# Autodesk Inventor assembly: DisceepXL
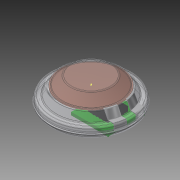
[picture p0: Inventor's stored thumbnail of the model, 180x180]
Saved by Autodesk Inventor 2014 (Build 180170000, 170)
## iProperties
Created: 2014-11-22
Part Number: DisceepXL
Document SubType Name: Assembly
Designer: DV
Author: DV
## Documents named in this file (8)
- C:\Users\DV\Documents\github\Disceep\DisceepXL.iam
- C:\Users\DV\Documents\github\Disceep\PAS614L-VL3.iam
- C:\Users\DV\Documents\github\Disceep\DisceepXL_PCB.ipt
- C:\Users\DV\Documents\github\Disceep\QFN16_4mmx4mm.ipt
- C:\Users\DV\Documents\github\Disceep\DisceepXL_Case.ipt
- C:\Users\DV\Documents\github\Disceep\12mmPiezo.ipt
- C:\Users\DV\Documents\github\Disceep\DisceepSL_CaseBottom.ipt
- C:\Users\DV\Documents\github\Disceep\Part3.ipt
## Components (7 placed, 7 different names)
1. PAS614L-VL3:1 [sub-assembly] — Mate:2, Mate:3, Mate:8
2. DisceepXL_PCB:1 — Mate:1, Mate:2, Mate:3, Mate:7, Mate:9, Angle:1
3. QFN16_4mmx4mm:1 — Mate:1, Flush:7, Mate:7
4. DisceepXL_Case:1 — Flush:9
5. 12mmPiezo:1 — Mate:4, Flush:6, Flush:7
6. DisceepSL_CaseBottom:1 — Flush:8
7. Part3:2 — Flush:9, Angle:1
## Relationships (12: Mate 7, Flush 4, Angle 1)
- Mate:1: DisceepXL_PCB:1 ↔ QFN16_4mmx4mm:1
- Mate:2: PAS614L-VL3:1 ↔ DisceepXL_PCB:1
- Mate:3 (0.254 mm): PAS614L-VL3:1 ↔ DisceepXL_PCB:1
- Mate:4: 12mmPiezo:1
- Flush:6: 12mmPiezo:1
- Flush:7 (1.905 mm): QFN16_4mmx4mm:1 ↔ 12mmPiezo:1
- Mate:7: DisceepXL_PCB:1 ↔ QFN16_4mmx4mm:1
- Mate:8: PAS614L-VL3:1
- Mate:9: DisceepXL_PCB:1
- Flush:8: DisceepSL_CaseBottom:1
- Flush:9: DisceepXL_Case:1 ↔ Part3:2
- Angle:1 (0 deg): DisceepXL_PCB:1 ↔ Part3:2
